# Autodesk Inventor assembly: ENSAMBLE_2
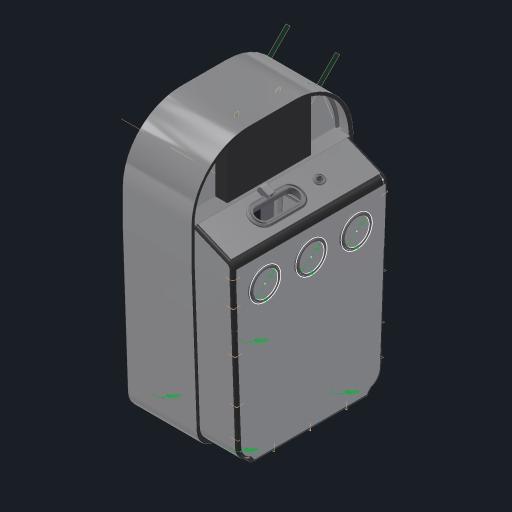
[picture p0: Inventor's stored thumbnail of the model, 512x512]
Saved by Autodesk Inventor 2024.3 (Build 283343000, 343)
## iProperties
Created: 2024-06-14
Part Number: ENSAMBLE_2
Material: Generic
Document SubType Name: Assembly
Designer: Niler
Author: Niler
## Documents named in this file (48)
- C:\Users\Niler\OneDrive\Escritorio\RECICLADOR\RECICLADOR_MODELO_3D\VERSION_3_COMPLETA\ENSAMBLE_2.iam
- C:\Users\Niler\OneDrive\Escritorio\RECICLADOR\RECICLADOR_MODELO_3D\VERSION_3_COMPLETA\CARCASA_ESTRUCTURA_Y_CHAPAS_2.iam
- C:\Users\Niler\OneDrive\Escritorio\RECICLADOR\RECICLADOR_MODELO_3D\VERSION_3_COMPLETA\PIEZAS_CHAPAS_ALUMINIO\CARCASA_ALUM_1.ipt
- C:\Users\Niler\OneDrive\Escritorio\RECICLADOR\RECICLADOR_MODELO_3D\VERSION_3_COMPLETA\ESQUINAS\ESQUINA_REDONDEADA_R20_P10.ipt
- C:\Users\Niler\OneDrive\Escritorio\RECICLADOR\RECICLADOR_MODELO_3D\VERSION_3_COMPLETA\ESQUINAS\ESQUINA_REDONDEADA_R20_P11.ipt
- C:\Users\Niler\OneDrive\Escritorio\RECICLADOR\RECICLADOR_MODELO_3D\VERSION_3_COMPLETA\ESQUINAS\ESQUINA_REDONDEADA_R20_P12.ipt
- C:\Users\Niler\OneDrive\Escritorio\RECICLADOR\RECICLADOR_MODELO_3D\VERSION_3_COMPLETA\NUEVAS_CHAPAS_ALUMINIO\CHAPA_1.ipt
- C:\Users\Niler\OneDrive\Escritorio\RECICLADOR\RECICLADOR_MODELO_3D\VERSION_3_COMPLETA\NUEVAS_CHAPAS_ALUMINIO\CHAPA_2.ipt
- C:\Users\Niler\OneDrive\Escritorio\RECICLADOR\RECICLADOR_MODELO_3D\VERSION_3_COMPLETA\NUEVAS_CHAPAS_ALUMINIO\CHAPA_3.ipt
- C:\Users\Niler\OneDrive\Escritorio\RECICLADOR\RECICLADOR_MODELO_3D\VERSION_3_COMPLETA\ESQUINAS\ESQUINA_REDONDEADA_R20_P5.ipt
- C:\Users\Niler\OneDrive\Escritorio\RECICLADOR\RECICLADOR_MODELO_3D\VERSION_3_COMPLETA\ESQUINAS\ESQUINA_REDONDEADA_R20_P13.ipt
- C:\Users\Niler\OneDrive\Escritorio\RECICLADOR\RECICLADOR_MODELO_3D\MECANISMO DE COMPACTADO\ENSAMBLE MECANISMO DE INGRESO.iam
- C:\Users\Niler\OneDrive\Escritorio\RECICLADOR\RECICLADOR_MODELO_3D\VERSION_3_COMPLETA\CURVA_SUPERIOR_IMPR.ipt
- C:\Users\Niler\OneDrive\Escritorio\RECICLADOR\RECICLADOR_MODELO_3D\VERSION_3_COMPLETA\ESQUINAS\ESQUINA_REDONDEADA_TRASERA.ipt
- C:\Users\Niler\OneDrive\Escritorio\RECICLADOR\RECICLADOR_MODELO_3D\VERSION_3_COMPLETA\ESQUINAS\ESQUINA_REDONDEADA_TRASERA_MIR.ipt
- C:\Users\Niler\OneDrive\Escritorio\RECICLADOR\RECICLADOR_MODELO_3D\VERSION_3_COMPLETA\CURVA_SUPERIOR_IMPR_MIR.ipt
- C:\Users\Niler\OneDrive\Escritorio\RECICLADOR\RECICLADOR_MODELO_3D\VERSION_3_COMPLETA\NUEVAS_CHAPAS_ALUMINIO\CHAPA_4_v2.ipt
- C:\Users\Niler\OneDrive\Escritorio\RECICLADOR\RECICLADOR_MODELO_3D\VERSION_3_COMPLETA\NUEVAS_CHAPAS_ALUMINIO\CHAPA_4_v2_MIR.ipt
- C:\Users\Niler\OneDrive\Escritorio\RECICLADOR\RECICLADOR_MODELO_3D\VERSION_3_COMPLETA\NUEVAS_CHAPAS_ALUMINIO\CHAPA_5.ipt
- C:\Users\Niler\OneDrive\Escritorio\RECICLADOR\RECICLADOR_MODELO_3D\VERSION_3_COMPLETA\ESQUINAS\ESQUINA_REDONDEADA_R20_P12_MIR.ipt
- C:\Users\Niler\OneDrive\Escritorio\RECICLADOR\RECICLADOR_MODELO_3D\VERSION_3_COMPLETA\NUEVAS_CHAPAS_ALUMINIO\CHAPA_6.ipt
- C:\Users\Niler\OneDrive\Escritorio\RECICLADOR\RECICLADOR_MODELO_3D\VERSION_3_COMPLETA\NUEVAS_CHAPAS_ALUMINIO\CHAPA_7.ipt
- C:\Users\Niler\OneDrive\Escritorio\RECICLADOR\RECICLADOR_MODELO_3D\VERSION_3_COMPLETA\CARCASA_PANTALLA.ipt
- C:\Users\Niler\OneDrive\Escritorio\RECICLADOR\RECICLADOR_MODELO_3D\VERSION_3_COMPLETA\PANTALLA.ipt
- C:\Users\Niler\OneDrive\Escritorio\RECICLADOR\RECICLADOR_MODELO_3D\VERSION_3_COMPLETA\ESQUINAS\ESQUINA_RECTA_SUPERIOR.ipt
- C:\Users\Niler\OneDrive\Escritorio\RECICLADOR\RECICLADOR_MODELO_3D\VERSION_3_COMPLETA\ESQUINAS\ESQUINA_RECTA_SUPERIOR_2.ipt
- C:\Users\Niler\OneDrive\Escritorio\RECICLADOR\RECICLADOR_MODELO_3D\VERSION_3_COMPLETA\NUEVAS_CHAPAS_ALUMINIO\CHAPA_7_MIR1.ipt
- C:\Users\Niler\OneDrive\Escritorio\RECICLADOR\RECICLADOR_MODELO_3D\VERSION_3_COMPLETA\ESQUINAS\ESQUINA_RECTA_SUPERIOR_MIR.ipt
- C:\Users\Niler\OneDrive\Escritorio\RECICLADOR\RECICLADOR_MODELO_3D\VERSION_3_COMPLETA\SEPARADOR.ipt
- C:\Users\Niler\OneDrive\Escritorio\RECICLADOR\RECICLADOR_MODELO_3D\VERSION_3_COMPLETA\SEPARADOR2.ipt
- C:\Users\Niler\OneDrive\Escritorio\RECICLADOR\RECICLADOR_MODELO_3D\VERSION_3_COMPLETA\SEPARADOR_3.ipt
- C:\Users\Niler\OneDrive\Escritorio\RECICLADOR\RECICLADOR_MODELO_3D\VERSION_3_COMPLETA\ESQUINAS\ESQUINA_REDONDEADA_TRASERA_MIR1.ipt
- C:\Users\Niler\OneDrive\Escritorio\RECICLADOR\RECICLADOR_MODELO_3D\VERSION_3_COMPLETA\SEPARADOR_MIR.ipt
- C:\Users\Niler\OneDrive\Escritorio\RECICLADOR\RECICLADOR_MODELO_3D\VERSION_3_COMPLETA\SEPARADOR2_MIR.ipt
- C:\Users\Niler\OneDrive\Escritorio\RECICLADOR\RECICLADOR_MODELO_3D\VERSION_3_COMPLETA\SEPARADOR4.ipt
- C:\Users\Niler\OneDrive\Escritorio\RECICLADOR\RECICLADOR_MODELO_3D\VERSION_3_COMPLETA\SEPARADOR_3_p2.ipt
- C:\Users\Niler\OneDrive\Escritorio\RECICLADOR\RECICLADOR_MODELO_3D\VERSION_3_COMPLETA\SEPARADOR_3_MIR1.ipt
- C:\Users\Niler\OneDrive\Escritorio\RECICLADOR\RECICLADOR_MODELO_3D\VERSION_3_COMPLETA\SEPARADOR_3_p2_MIR.ipt
- C:\Users\Niler\OneDrive\Escritorio\RECICLADOR\RECICLADOR_MODELO_3D\VERSION_3_COMPLETA\NUEVAS_CHAPAS_ALUMINIO\CHAPA_9.ipt
- C:\Users\Niler\OneDrive\Escritorio\RECICLADOR\RECICLADOR_MODELO_3D\VERSION_3_COMPLETA\COMPUERTA_PLASTICO.ipt
- C:\Users\Niler\OneDrive\Escritorio\RECICLADOR\RECICLADOR_MODELO_3D\VERSION_3_COMPLETA\ESQUINERO_PUERTAS.ipt
- C:\Users\Niler\OneDrive\Escritorio\RECICLADOR\RECICLADOR_MODELO_3D\VERSION_3_COMPLETA\COMPUERTA_CHAPAS_PLASTICO.ipt
- C:\Users\Niler\OneDrive\Escritorio\RECICLADOR\RECICLADOR_MODELO_3D\VERSION_3_COMPLETA\PATA_PLASTICO.ipt
- C:\Users\Niler\OneDrive\Escritorio\RECICLADOR\RECICLADOR_MODELO_3D\CIRCULO_fRONTAL.ipt
- C:\Users\Niler\OneDrive\Escritorio\RECICLADOR\RECICLADOR_MODELO_3D\DOOR_HANDLE.ipt
- C:\Users\Niler\OneDrive\Escritorio\RECICLADOR\RECICLADOR_MODELO_3D\VERSION_3_COMPLETA\ESQUINERO_PUERTAS_MIR.ipt
- C:\Users\Niler\OneDrive\Escritorio\RECICLADOR\RECICLADOR_MODELO_3D\soporte_sensor_puerta.ipt
- C:\Users\Niler\OneDrive\Escritorio\RECICLADOR\RECICLADOR_MODELO_3D\INFRARROJO.ipt
## Components (72 placed, 47 different names)
1. CARCASA_ESTRUCTURA_Y_CHAPAS_2:1 [sub-assembly] — Flush:1, Mate:2, Mate:3, Mate:6, Mate:13, Mate:14, Mate:15, Mate:17, Mate:21, Mate:22, Mate:23, Mate:30, Mate:31, Mate:32, Mate:33, Mate:34, Mate:35, Mate:38, Mate:39, Flush:12, Mate:40, Flush:16, Mate:45, Flush:17, Mate:46, Mate:50, Mate:51, Flush:18, Flush:20, Flush:21, Mate:55, Mate:56, Mate:58, Mate:59, Mate:60, Mate:61, Mate:62, Mate:63, Mate:64, Mate:65, Mate:66, Flush:48, Flush:49, Flush:50, Mate:105, Mate:106
2. CARCASA_ALUM_1:1 — Flush:1, Mate:40, Mate:41, Mate:53, Mate:71, Flush:28, Mate:83
3. ESQUINA_REDONDEADA_R20_P10:1 — Mate:2, Mate:4, Mate:5, Mate:6, Mate:9, Flush:2, Mate:16
4. ESQUINA_REDONDEADA_R20_P11:1 — Mate:3, Mate:4, Mate:5, Mate:36
5. ESQUINA_REDONDEADA_R20_P10:2 — Mate:9, Flush:2, Flush:5, Mate:12, Flush:11
6. ESQUINA_REDONDEADA_R20_P11:2 — Flush:11, Mate:36, Mate:37
7. ESQUINA_REDONDEADA_R20_P10:3 — Flush:5, Mate:12
8. ESQUINA_REDONDEADA_R20_P11:3 — Mate:37, Mate:103
9. ESQUINA_REDONDEADA_R20_P12:1 — Mate:13, Mate:14, Mate:15, Mate:57
10. CHAPA_1:1 — Mate:33, Mate:34, Mate:35, Mate:97, Mate:98, Mate:102, Flush:51, Flush:52
11. CHAPA_2:1 — Mate:18, Flush:6, Mate:107, Mate:108, Mate:109
12. CHAPA_3:1 — Mate:16, Mate:17, Mate:18, Flush:6
13. ESQUINA_REDONDEADA_R20_P5:1 — Mate:22, Mate:27
14. ESQUINA_REDONDEADA_R20_P5:2 — Mate:21, Mate:23, Mate:26, Flush:9
15. ESQUINA_REDONDEADA_R20_P5:3 — Mate:27
16. ESQUINA_REDONDEADA_R20_P5:4 — Mate:26, Flush:9
17. ESQUINA_REDONDEADA_R20_P13:1 — Mate:28, Flush:10, Mate:29, Mate:30
18. ESQUINA_REDONDEADA_R20_P13:2 — Mate:28, Flush:10, Mate:29, Mate:31, Mate:32
19. ENSAMBLE MECANISMO DE INGRESO:1 [sub-assembly] — Mate:38, Mate:39
20. CURVA_SUPERIOR_IMPR:1 — Flush:12, Mate:41, Mate:44, Mate:47
21. CURVA_SUPERIOR_IMPR:3 — Mate:44, Flush:16, Mate:47, Flush:19
22. ESQUINA_REDONDEADA_TRASERA:1 — Mate:45, Flush:17, Mate:46, Mate:52
23. ESQUINA_REDONDEADA_TRASERA_MIR:1
24. CURVA_SUPERIOR_IMPR_MIR:1 — Mate:48, Mate:49
25. CURVA_SUPERIOR_IMPR_MIR:2 — Mate:48, Mate:49
26. CHAPA_4_v2:1 — Mate:50, Mate:51, Mate:69
27. CHAPA_4_v2_MIR:1
28. CHAPA_5:1 — Mate:52, Flush:18, Mate:53
29. ESQUINA_REDONDEADA_R20_P12_MIR:1 — Mate:104
30. CHAPA_6:1 — Flush:19, Mate:99, Mate:100, Mate:101
31. CHAPA_7:1 — Flush:20, Flush:21
32. CARCASA_PANTALLA:1 — Mate:55, Mate:96
33. PANTALLA:1 — Mate:56
34. ESQUINA_REDONDEADA_TRASERA:2 — Mate:57, Mate:58, Mate:59, Flush:22, Mate:67
35. ESQUINA_RECTA_SUPERIOR:1 — Mate:60, Mate:61, Mate:62, Mate:94, Flush:47
36. ESQUINA_RECTA_SUPERIOR_2:1 — Mate:63, Mate:64
37. ESQUINA_RECTA_SUPERIOR_2:2 — Mate:65, Mate:66
38. CHAPA_7_MIR1:1
39. ESQUINA_RECTA_SUPERIOR_MIR:1
40. SEPARADOR:1 — Flush:22, Mate:67, Mate:68, Flush:23, Flush:24, Mate:69
41. SEPARADOR:2 — Mate:68, Flush:23, Flush:24, Flush:25, Flush:26, Mate:70
42. SEPARADOR:3 — Flush:25, Flush:26, Mate:70, Mate:73, Flush:27
43. SEPARADOR2:1 — Mate:71, Mate:73, Flush:27
44. SEPARADOR_3:1 — Flush:28, Flush:38, Flush:39, Mate:84, Mate:85, Flush:41, Flush:42, Mate:95
45. ESQUINA_REDONDEADA_TRASERA_MIR1:1 — Mate:77, Flush:31
46. SEPARADOR_MIR:1 — Mate:77, Flush:31, Flush:32, Flush:33, Mate:78
47. SEPARADOR_MIR:2 — Flush:32, Flush:33, Mate:78, Mate:79, Flush:34, Flush:35
48. SEPARADOR_MIR:3 — Mate:79, Flush:34, Flush:35, Flush:36, Mate:80
49. SEPARADOR2_MIR:1 — Flush:36, Mate:80
50. SEPARADOR4:1 — Mate:83, Flush:38
51. SEPARADOR_3_p2:1 — Flush:39, Mate:84, Mate:85, Mate:88
52. SEPARADOR_3:2 — Flush:41
53. SEPARADOR_3_p2:2 — Flush:42, Mate:88
54. SEPARADOR_3_MIR1:1 — Mate:89, Mate:90, Flush:43, Flush:44, Flush:45
55. SEPARADOR_3_p2_MIR:1 — Mate:89, Mate:90, Flush:43, Mate:91
56. SEPARADOR_3_MIR1:2 — Flush:44, Mate:92, Mate:93, Flush:46
57. SEPARADOR_3_p2_MIR:2 — Flush:45, Mate:91, Mate:92, Mate:93, Flush:46
58. CHAPA_9:1 — Mate:94, Mate:95, Flush:47, Mate:96
59. COMPUERTA_PLASTICO:1 — Mate:97, Mate:98
60. ESQUINERO_PUERTAS:1 — Mate:99, Mate:100, Mate:101
61. COMPUERTA_CHAPAS_PLASTICO:1 — Mate:102
62. PATA_PLASTICO:1 — Flush:50, Mate:105, Mate:106
63. PATA_PLASTICO:2 — Flush:48
64. PATA_PLASTICO:3 — Flush:49, Mate:103, Mate:104
65. PATA_PLASTICO:4
66. CIRCULO_fRONTAL:1 — Mate:107
67. CIRCULO_fRONTAL:2 — Mate:108
68. CIRCULO_fRONTAL:3 — Mate:109
69. DOOR_HANDLE:1
70. ESQUINERO_PUERTAS_MIR:1
71. soporte_sensor_puerta:1 — Flush:51, Flush:52, Mate:110, Flush:53
72. INFRARROJO:1 — Mate:110, Flush:53
## Relationships (145: Mate 100, Flush 45)
- Flush:1: CARCASA_ESTRUCTURA_Y_CHAPAS_2:1 ↔ CARCASA_ALUM_1:1
- Mate:2: CARCASA_ESTRUCTURA_Y_CHAPAS_2:1 ↔ ESQUINA_REDONDEADA_R20_P10:1
- Mate:3: CARCASA_ESTRUCTURA_Y_CHAPAS_2:1 ↔ ESQUINA_REDONDEADA_R20_P11:1
- Mate:4: ESQUINA_REDONDEADA_R20_P10:1 ↔ ESQUINA_REDONDEADA_R20_P11:1
- Mate:5: ESQUINA_REDONDEADA_R20_P10:1 ↔ ESQUINA_REDONDEADA_R20_P11:1
- Mate:6: CARCASA_ESTRUCTURA_Y_CHAPAS_2:1 ↔ ESQUINA_REDONDEADA_R20_P10:1
- [Mate]: ESQUINA_REDONDEADA_R20_P10:2 ↔ ESQUINA_REDONDEADA_R20_P11:2
- [Mate]: ESQUINA_REDONDEADA_R20_P10:2 ↔ ESQUINA_REDONDEADA_R20_P11:2
- Mate:9: ESQUINA_REDONDEADA_R20_P10:1 ↔ ESQUINA_REDONDEADA_R20_P10:2
- Flush:2: ESQUINA_REDONDEADA_R20_P10:1 ↔ ESQUINA_REDONDEADA_R20_P10:2
- [Mate]: ESQUINA_REDONDEADA_R20_P10:3 ↔ ESQUINA_REDONDEADA_R20_P11:3
- [Mate]: ESQUINA_REDONDEADA_R20_P10:3 ↔ ESQUINA_REDONDEADA_R20_P11:3
- Flush:5: ESQUINA_REDONDEADA_R20_P10:2 ↔ ESQUINA_REDONDEADA_R20_P10:3
- Mate:12: ESQUINA_REDONDEADA_R20_P10:2 ↔ ESQUINA_REDONDEADA_R20_P10:3
- Mate:13: CARCASA_ESTRUCTURA_Y_CHAPAS_2:1 ↔ ESQUINA_REDONDEADA_R20_P12:1
- Mate:14: CARCASA_ESTRUCTURA_Y_CHAPAS_2:1 ↔ ESQUINA_REDONDEADA_R20_P12:1
- Mate:15: CARCASA_ESTRUCTURA_Y_CHAPAS_2:1 ↔ ESQUINA_REDONDEADA_R20_P12:1
- Mate:16: ESQUINA_REDONDEADA_R20_P10:1 ↔ CHAPA_3:1
- Mate:17: CARCASA_ESTRUCTURA_Y_CHAPAS_2:1 ↔ CHAPA_3:1
- Mate:18: CHAPA_2:1 ↔ CHAPA_3:1
- Flush:6: CHAPA_2:1 ↔ CHAPA_3:1
- [Mate]: ESQUINA_REDONDEADA_R20_P5:1 ↔ ESQUINA_REDONDEADA_R20_P5:2
- [Flush]: ESQUINA_REDONDEADA_R20_P5:1 ↔ ESQUINA_REDONDEADA_R20_P5:2
- [Mate]: ESQUINA_REDONDEADA_R20_P5:1 ↔ ESQUINA_REDONDEADA_R20_P5:2
- Mate:21: CARCASA_ESTRUCTURA_Y_CHAPAS_2:1 ↔ ESQUINA_REDONDEADA_R20_P5:2
- Mate:22: CARCASA_ESTRUCTURA_Y_CHAPAS_2:1 ↔ ESQUINA_REDONDEADA_R20_P5:1
- Mate:23: CARCASA_ESTRUCTURA_Y_CHAPAS_2:1 ↔ ESQUINA_REDONDEADA_R20_P5:2
- [Mate]: ESQUINA_REDONDEADA_R20_P5:3 ↔ ESQUINA_REDONDEADA_R20_P5:4
- [Flush]: ESQUINA_REDONDEADA_R20_P5:3 ↔ ESQUINA_REDONDEADA_R20_P5:4
- [Mate]: ESQUINA_REDONDEADA_R20_P5:3 ↔ ESQUINA_REDONDEADA_R20_P5:4
- Mate:26: ESQUINA_REDONDEADA_R20_P5:2 ↔ ESQUINA_REDONDEADA_R20_P5:4
- Mate:27: ESQUINA_REDONDEADA_R20_P5:1 ↔ ESQUINA_REDONDEADA_R20_P5:3
- Flush:9: ESQUINA_REDONDEADA_R20_P5:2 ↔ ESQUINA_REDONDEADA_R20_P5:4
- Mate:28: ESQUINA_REDONDEADA_R20_P13:1 ↔ ESQUINA_REDONDEADA_R20_P13:2
- Flush:10: ESQUINA_REDONDEADA_R20_P13:1 ↔ ESQUINA_REDONDEADA_R20_P13:2
- Mate:29: ESQUINA_REDONDEADA_R20_P13:1 ↔ ESQUINA_REDONDEADA_R20_P13:2
- Mate:30: CARCASA_ESTRUCTURA_Y_CHAPAS_2:1 ↔ ESQUINA_REDONDEADA_R20_P13:1
- Mate:31: CARCASA_ESTRUCTURA_Y_CHAPAS_2:1 ↔ ESQUINA_REDONDEADA_R20_P13:2
- Mate:32: CARCASA_ESTRUCTURA_Y_CHAPAS_2:1 ↔ ESQUINA_REDONDEADA_R20_P13:2
- Mate:33: CARCASA_ESTRUCTURA_Y_CHAPAS_2:1 ↔ CHAPA_1:1
- Mate:34: CARCASA_ESTRUCTURA_Y_CHAPAS_2:1 ↔ CHAPA_1:1
- Mate:35: CARCASA_ESTRUCTURA_Y_CHAPAS_2:1 ↔ CHAPA_1:1
- Flush:11: ESQUINA_REDONDEADA_R20_P10:2 ↔ ESQUINA_REDONDEADA_R20_P11:2
- Mate:36: ESQUINA_REDONDEADA_R20_P11:1 ↔ ESQUINA_REDONDEADA_R20_P11:2
- Mate:37: ESQUINA_REDONDEADA_R20_P11:2 ↔ ESQUINA_REDONDEADA_R20_P11:3
- Mate:38: CARCASA_ESTRUCTURA_Y_CHAPAS_2:1 ↔ ENSAMBLE MECANISMO DE INGRESO:1
- Mate:39 (5 mm): CARCASA_ESTRUCTURA_Y_CHAPAS_2:1 ↔ ENSAMBLE MECANISMO DE INGRESO:1
- Flush:12: CARCASA_ESTRUCTURA_Y_CHAPAS_2:1 ↔ CURVA_SUPERIOR_IMPR:1
- Mate:40: CARCASA_ESTRUCTURA_Y_CHAPAS_2:1 ↔ CARCASA_ALUM_1:1
- Mate:41: CARCASA_ALUM_1:1 ↔ CURVA_SUPERIOR_IMPR:1
- Mate:44: CURVA_SUPERIOR_IMPR:1 ↔ CURVA_SUPERIOR_IMPR:3
- Flush:16: CARCASA_ESTRUCTURA_Y_CHAPAS_2:1 ↔ CURVA_SUPERIOR_IMPR:3
- Mate:45: CARCASA_ESTRUCTURA_Y_CHAPAS_2:1 ↔ ESQUINA_REDONDEADA_TRASERA:1
- Flush:17: CARCASA_ESTRUCTURA_Y_CHAPAS_2:1 ↔ ESQUINA_REDONDEADA_TRASERA:1
- Mate:46: CARCASA_ESTRUCTURA_Y_CHAPAS_2:1 ↔ ESQUINA_REDONDEADA_TRASERA:1
- Mate:47: CURVA_SUPERIOR_IMPR:1 ↔ CURVA_SUPERIOR_IMPR:3
- Mate:48: CURVA_SUPERIOR_IMPR_MIR:1 ↔ CURVA_SUPERIOR_IMPR_MIR:2
- Mate:49: CURVA_SUPERIOR_IMPR_MIR:1 ↔ CURVA_SUPERIOR_IMPR_MIR:2
- Mate:50: CARCASA_ESTRUCTURA_Y_CHAPAS_2:1 ↔ CHAPA_4_v2:1
- Mate:51: CARCASA_ESTRUCTURA_Y_CHAPAS_2:1 ↔ CHAPA_4_v2:1
- Mate:52: ESQUINA_REDONDEADA_TRASERA:1 ↔ CHAPA_5:1
- Flush:18: CARCASA_ESTRUCTURA_Y_CHAPAS_2:1 ↔ CHAPA_5:1
- Mate:53: CARCASA_ALUM_1:1 ↔ CHAPA_5:1
- Flush:19: CURVA_SUPERIOR_IMPR:3 ↔ CHAPA_6:1
- Flush:20: CARCASA_ESTRUCTURA_Y_CHAPAS_2:1 ↔ CHAPA_7:1
- Flush:21: CARCASA_ESTRUCTURA_Y_CHAPAS_2:1 ↔ CHAPA_7:1
- Mate:55: CARCASA_ESTRUCTURA_Y_CHAPAS_2:1 ↔ CARCASA_PANTALLA:1
- Mate:56: CARCASA_ESTRUCTURA_Y_CHAPAS_2:1 ↔ PANTALLA:1
- Mate:57: ESQUINA_REDONDEADA_R20_P12:1 ↔ ESQUINA_REDONDEADA_TRASERA:2
- Mate:58: CARCASA_ESTRUCTURA_Y_CHAPAS_2:1 ↔ ESQUINA_REDONDEADA_TRASERA:2
- Mate:59: CARCASA_ESTRUCTURA_Y_CHAPAS_2:1 ↔ ESQUINA_REDONDEADA_TRASERA:2
- Mate:60: CARCASA_ESTRUCTURA_Y_CHAPAS_2:1 ↔ ESQUINA_RECTA_SUPERIOR:1
- Mate:61: CARCASA_ESTRUCTURA_Y_CHAPAS_2:1 ↔ ESQUINA_RECTA_SUPERIOR:1
- Mate:62: CARCASA_ESTRUCTURA_Y_CHAPAS_2:1 ↔ ESQUINA_RECTA_SUPERIOR:1
- Mate:63: CARCASA_ESTRUCTURA_Y_CHAPAS_2:1 ↔ ESQUINA_RECTA_SUPERIOR_2:1
- Mate:64: CARCASA_ESTRUCTURA_Y_CHAPAS_2:1 ↔ ESQUINA_RECTA_SUPERIOR_2:1
- Mate:65: CARCASA_ESTRUCTURA_Y_CHAPAS_2:1 ↔ ESQUINA_RECTA_SUPERIOR_2:2
- Mate:66: CARCASA_ESTRUCTURA_Y_CHAPAS_2:1 ↔ ESQUINA_RECTA_SUPERIOR_2:2
- Flush:22: ESQUINA_REDONDEADA_TRASERA:2 ↔ SEPARADOR:1
- Mate:67: ESQUINA_REDONDEADA_TRASERA:2 ↔ SEPARADOR:1
- Mate:68: SEPARADOR:1 ↔ SEPARADOR:2
- Flush:23: SEPARADOR:1 ↔ SEPARADOR:2
- Flush:24: SEPARADOR:1 ↔ SEPARADOR:2
- Mate:69: CHAPA_4_v2:1 ↔ SEPARADOR:1
- Flush:25: SEPARADOR:2 ↔ SEPARADOR:3
- Flush:26: SEPARADOR:2 ↔ SEPARADOR:3
- Mate:70: SEPARADOR:2 ↔ SEPARADOR:3
- Mate:71: CARCASA_ALUM_1:1 ↔ SEPARADOR2:1
- Mate:73: SEPARADOR:3 ↔ SEPARADOR2:1
- Flush:27: SEPARADOR:3 ↔ SEPARADOR2:1
- Flush:28: CARCASA_ALUM_1:1 ↔ SEPARADOR_3:1
- Mate:77: ESQUINA_REDONDEADA_TRASERA_MIR1:1 ↔ SEPARADOR_MIR:1
- Flush:31: ESQUINA_REDONDEADA_TRASERA_MIR1:1 ↔ SEPARADOR_MIR:1
- Flush:32: SEPARADOR_MIR:1 ↔ SEPARADOR_MIR:2
- Flush:33: SEPARADOR_MIR:1 ↔ SEPARADOR_MIR:2
- Mate:78: SEPARADOR_MIR:1 ↔ SEPARADOR_MIR:2
- Mate:79: SEPARADOR_MIR:2 ↔ SEPARADOR_MIR:3
- Flush:34: SEPARADOR_MIR:2 ↔ SEPARADOR_MIR:3
- Flush:35: SEPARADOR_MIR:2 ↔ SEPARADOR_MIR:3
- Flush:36: SEPARADOR_MIR:3 ↔ SEPARADOR2_MIR:1
- Mate:80: SEPARADOR_MIR:3 ↔ SEPARADOR2_MIR:1
- Mate:83: CARCASA_ALUM_1:1 ↔ SEPARADOR4:1
- Flush:38: SEPARADOR_3:1 ↔ SEPARADOR4:1
- Flush:39: SEPARADOR_3:1 ↔ SEPARADOR_3_p2:1
- Mate:84: SEPARADOR_3:1 ↔ SEPARADOR_3_p2:1
- Mate:85: SEPARADOR_3:1 ↔ SEPARADOR_3_p2:1
- [Flush]: SEPARADOR_3:2 ↔ SEPARADOR_3_p2:2
- [Mate]: SEPARADOR_3:2 ↔ SEPARADOR_3_p2:2
- [Mate]: SEPARADOR_3:2 ↔ SEPARADOR_3_p2:2
- Flush:41: SEPARADOR_3:1 ↔ SEPARADOR_3:2
- Flush:42 (90 mm): SEPARADOR_3:1 ↔ SEPARADOR_3_p2:2
- Mate:88: SEPARADOR_3_p2:1 ↔ SEPARADOR_3_p2:2
- Mate:89: SEPARADOR_3_MIR1:1 ↔ SEPARADOR_3_p2_MIR:1
- Mate:90: SEPARADOR_3_MIR1:1 ↔ SEPARADOR_3_p2_MIR:1
- Flush:43: SEPARADOR_3_MIR1:1 ↔ SEPARADOR_3_p2_MIR:1
- Flush:44: SEPARADOR_3_MIR1:1 ↔ SEPARADOR_3_MIR1:2
- Flush:45 (90 mm): SEPARADOR_3_MIR1:1 ↔ SEPARADOR_3_p2_MIR:2
- Mate:91: SEPARADOR_3_p2_MIR:1 ↔ SEPARADOR_3_p2_MIR:2
- Mate:92: SEPARADOR_3_MIR1:2 ↔ SEPARADOR_3_p2_MIR:2
- Mate:93: SEPARADOR_3_MIR1:2 ↔ SEPARADOR_3_p2_MIR:2
- Flush:46: SEPARADOR_3_MIR1:2 ↔ SEPARADOR_3_p2_MIR:2
- Mate:94: ESQUINA_RECTA_SUPERIOR:1 ↔ CHAPA_9:1
- Mate:95: SEPARADOR_3:1 ↔ CHAPA_9:1
- Flush:47: ESQUINA_RECTA_SUPERIOR:1 ↔ CHAPA_9:1
- Mate:96: CARCASA_PANTALLA:1 ↔ CHAPA_9:1
- Mate:97: CHAPA_1:1 ↔ COMPUERTA_PLASTICO:1
- Mate:98: CHAPA_1:1 ↔ COMPUERTA_PLASTICO:1
- Mate:99: CHAPA_6:1 ↔ ESQUINERO_PUERTAS:1
- Mate:100: CHAPA_6:1 ↔ ESQUINERO_PUERTAS:1
- Mate:101: CHAPA_6:1 ↔ ESQUINERO_PUERTAS:1
- Mate:102: CHAPA_1:1 ↔ COMPUERTA_CHAPAS_PLASTICO:1
- Flush:48: CARCASA_ESTRUCTURA_Y_CHAPAS_2:1 ↔ PATA_PLASTICO:2
- Flush:49: CARCASA_ESTRUCTURA_Y_CHAPAS_2:1 ↔ PATA_PLASTICO:3
- Mate:103: ESQUINA_REDONDEADA_R20_P11:3 ↔ PATA_PLASTICO:3
- Mate:104: ESQUINA_REDONDEADA_R20_P12_MIR:1 ↔ PATA_PLASTICO:3
- Flush:50: CARCASA_ESTRUCTURA_Y_CHAPAS_2:1 ↔ PATA_PLASTICO:1
- Mate:105: CARCASA_ESTRUCTURA_Y_CHAPAS_2:1 ↔ PATA_PLASTICO:1
- Mate:106: CARCASA_ESTRUCTURA_Y_CHAPAS_2:1 ↔ PATA_PLASTICO:1
- Mate:107: CHAPA_2:1 ↔ CIRCULO_fRONTAL:1
- Mate:108: CHAPA_2:1 ↔ CIRCULO_fRONTAL:2
- Mate:109: CHAPA_2:1 ↔ CIRCULO_fRONTAL:3
- Flush:51: CHAPA_1:1 ↔ soporte_sensor_puerta:1
- Flush:52: CHAPA_1:1 ↔ soporte_sensor_puerta:1
- Mate:110: soporte_sensor_puerta:1 ↔ INFRARROJO:1
- Flush:53: soporte_sensor_puerta:1 ↔ INFRARROJO:1
## Named parameters: d8_d4 = 0 mm, d9_d5 = 0 mm, d13_d4 = 0 mm, d14_d5 = 0 mm, d38_d186 = 0 mm, d39_d187 = 0 mm, d40_d188 = 0 mm, d149_d146 = 0 mm, d150_d147 = 0 mm, d151_d148 = 0 mm
